# Autodesk Inventor assembly: 3D_Print_Chasis_FIXED
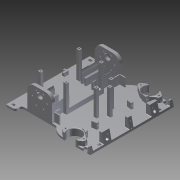
[picture p0: Inventor's stored thumbnail of the model, 180x180]
Saved by Autodesk Inventor 2011 SP2 (Build 150309200, 309)
## iProperties
Created: 2015-11-08
Part Number: 3D_Print_Chasis_FIXED
Document SubType Name: Assembly
Designer: Ernest
Author: Ernest
## Documents named in this file (2)
- D:\Inventor\Sumobot_3rd_Year\3D_Printing\3D_Print_Chasis_FIXED.iam
- D:\Inventor\Sumobot_3rd_Year\Chassis.ipt
## Components (1 placed, 1 different names)
1. Chassis:1 — Mate:1, Mate:2, Mate:3
## Relationships (3: Mate 3)
- Mate:1: Chassis:1
- Mate:2 (-75.5 mm): Chassis:1
- Mate:3 (-90 mm): Chassis:1
